# Autodesk Inventor assembly: ChargingArmAssembly
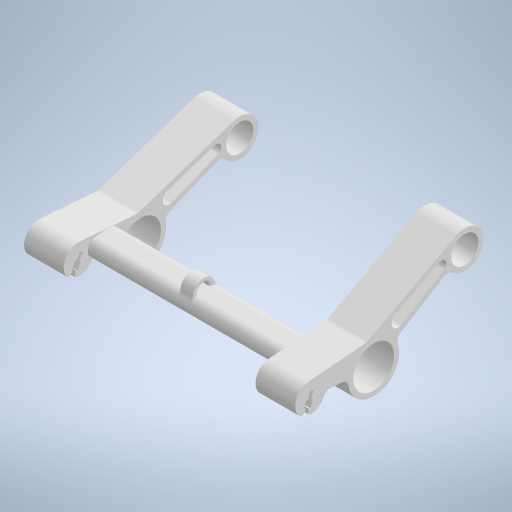
[picture p0: Inventor's stored thumbnail of the model, 512x512]
Saved by Autodesk Inventor 2023 (Build 270158000, 158)
## iProperties
Created: 2023-03-29
Part Number: ChargingArmAssembly
Document SubType Name: Assembly
Designer: Administrator
Author: Administrator
## Documents named in this file (3)
- C:\Users\Administrator\Documents\GitHub\WU-Team20-AutonomousDrone\CAD\Legs\ChargingArmAssembly.iam
- C:\Users\Administrator\Documents\GitHub\WU-Team20-AutonomousDrone\CAD\Legs\ChargingArm.ipt
- C:\Users\Administrator\Documents\GitHub\WU-Team20-AutonomousDrone\CAD\Legs\ChargingArm - ConnectingBrace.ipt
## Components (3 placed, 2 different names)
1. ChargingArm:1 — Rigid:2
2. ChargingArm:2 — Rigid:1
3. ChargingArm - ConnectingBrace:1 — Rigid:1, Rigid:2
## Relationships (2: WeldJoint 2)
- Rigid:1 [WeldJoint]: ChargingArm:2 ↔ ChargingArm - ConnectingBrace:1
- Rigid:2 [WeldJoint]: ChargingArm:1 ↔ ChargingArm - ConnectingBrace:1
